# Autodesk Inventor assembly: V5PCB 1
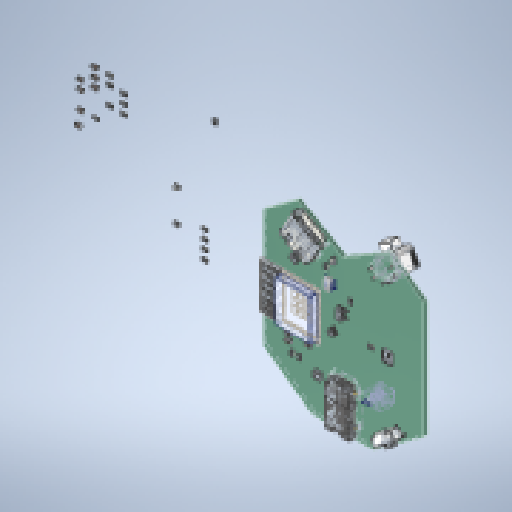
[picture p0: Inventor's stored thumbnail of the model, 512x512]
Saved by Autodesk Inventor 2024 (Build 280153000, 153)
## iProperties
Company: Kicad
Created: 2023-11-12
Part Number: V5PCB 1
Description: KiCad electronic assembly
Document SubType Name: Assembly
Designer: jevan
Authority: Unknown
Sending System: KiCad to STEP converter
Preprocessor: Open CASCADE STEP processor 7.7
Title: V5PCB.step
Author: Pcbnew
## Documents named in this file (17)
- D:\Windows.old.000\Users\jevan\Documents\Models\Lilypad\V5\V5PCB\V5PCB\V5PCB.iam
- D:\Windows.old.000\Users\jevan\Documents\Models\Lilypad\V5\V5PCB\V5PCB\R_0603_1608Metric.iam
- D:\Windows.old.000\Users\jevan\Documents\Models\Lilypad\V5\V5PCB\V5PCB\SW-SMD_YTSB001XXXX.iam
- D:\Windows.old.000\Users\jevan\Documents\Models\Lilypad\V5\V5PCB\V5PCB\C_0603_1608Metric.iam
- D:\Windows.old.000\Users\jevan\Documents\Models\Lilypad\V5\V5PCB\V5PCB\LED_0603_1608Metric.iam
- D:\Windows.old.000\Users\jevan\Documents\Models\Lilypad\V5\V5PCB\V5PCB\AUDIO-TH_ST-0277D00-052-142.iam
- D:\Windows.old.000\Users\jevan\Documents\Models\Lilypad\V5\V5PCB\V5PCB\L_0603_1608Metric.iam
- D:\Windows.old.000\Users\jevan\Documents\Models\Lilypad\V5\V5PCB\V5PCB\SOT-363_SC-70-6.iam
- D:\Windows.old.000\Users\jevan\Documents\Models\Lilypad\V5\V5PCB\V5PCB\Bosch_LGA-14_3x2.5mm_P0.5mm.iam
- D:\Windows.old.000\Users\jevan\Documents\Models\Lilypad\V5\V5PCB\V5PCB\DFN-8_L2.0-W2.0-P0.50-BL-EP.iam
- D:\Windows.old.000\Users\jevan\Documents\Models\Lilypad\V5\V5PCB\V5PCB\ESP32-C3-MINI-1-N4.iam
- D:\Windows.old.000\Users\jevan\Documents\Models\Lilypad\V5\V5PCB\V5PCB\BQ21040DBVR.iam
- D:\Windows.old.000\Users\jevan\Documents\Models\Lilypad\V5\V5PCB\V5PCB\SOT-23-5.iam
- D:\Windows.old.000\Users\jevan\Documents\Models\Lilypad\V5\V5PCB\V5PCB\USB_C_Receptacle_GCT_USB4105-xx-A_16P_TopMnt_Horizontal.iam
- D:\Windows.old.000\Users\jevan\Documents\Models\Lilypad\V5\V5PCB\V5PCB\SW-TH_TK-6580A8-1.iam
- D:\Windows.old.000\Users\jevan\Documents\Models\Lilypad\V5\V5PCB\V5PCB\CONN-TH_0530470210.iam
- D:\Windows.old.000\Users\jevan\Documents\Models\Lilypad\V5\V5PCB\V5PCB\V5PCB PCB.ipt
## Components (45 placed, 45 different names)
1. 2 [sub-assembly]
2. 4 [sub-assembly]
3. 6 [sub-assembly]
4. 7 [sub-assembly]
5. 9 [sub-assembly]
6. 10 [sub-assembly]
7. 11 [sub-assembly]
8. 12 [sub-assembly]
9. 14 [sub-assembly]
10. 15 [sub-assembly]
11. 16 [sub-assembly]
12. 17 [sub-assembly]
13. 18 [sub-assembly]
14. 19 [sub-assembly]
15. 21 [sub-assembly]
16. 22 [sub-assembly]
17. 23 [sub-assembly]
18. 24 [sub-assembly]
19. 25 [sub-assembly]
20. 26 [sub-assembly]
21. 27 [sub-assembly]
22. 28 [sub-assembly]
23. 29 [sub-assembly]
24. 31 [sub-assembly]
25. 33 [sub-assembly]
26. 34 [sub-assembly]
27. 36 [sub-assembly]
28. 37 [sub-assembly]
29. 39 [sub-assembly]
30. 40 [sub-assembly]
31. 41 [sub-assembly]
32. 43 [sub-assembly]
33. 44 [sub-assembly]
34. 45 [sub-assembly]
35. 46 [sub-assembly]
36. 47 [sub-assembly]
37. 48 [sub-assembly]
38. 49 [sub-assembly]
39. 50 [sub-assembly]
40. 52 [sub-assembly]
41. 54 [sub-assembly]
42. 55 [sub-assembly]
43. 57 [sub-assembly] — Mate:2, Flush:1
44. 59 [sub-assembly] — Mate:1
45. 60 — Mate:1, Mate:2, Flush:1
## Relationships (3: Mate 2, Flush 1)
- Mate:1: 59 ↔ 60
- Mate:2 (6.874 mm): 57 ↔ 60
- Flush:1 (0.7 mm): 57 ↔ 60
